# Autodesk Inventor assembly: POM_T5_11
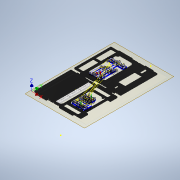
[picture p0: Inventor's stored thumbnail of the model, 180x180]
Saved by Autodesk Inventor 2020 (Build 240168000, 168)
## iProperties
Created: 2021-08-27
Part Number: POM_T5_11
Document SubType Name: Assembly
Designer: Masato
Author: Masato
## Documents named in this file (15)
- C:\Users\L20C1118 森　圭汰\Documents\220428_open\SUSTAINA-OP\Cam\POM_T5_11.iam
- C:\Users\L20C1118 森　圭汰\Documents\220428_open\SUSTAINA-OP\Cam\DisposableBoard.ipt
- C:\Users\L20C1118 森　圭汰\Documents\220428_open\SUSTAINA-OP\UpperBody\Cockpit\Cockpit_carrier_board_frame.ipt
- C:\Users\L20C1118 森　圭汰\Documents\220428_open\SUSTAINA-OP\UpperBody\Cockpit\Cockpit_circuit_board_frame.ipt
- C:\Users\L20C1118 森　圭汰\Documents\220428_open\SUSTAINA-OP\UpperBody\Cockpit\Cockpit_front_frame.ipt
- C:\Users\L20C1118 森　圭汰\Documents\220428_open\SUSTAINA-OP\Jig\Head_horn_frame_Jig.ipt
- C:\Users\L20C1118 森　圭汰\Documents\220428_open\SUSTAINA-OP\UpperBody\Cockpit\Cockpit_back_frame.ipt
- C:\Users\L20C1118 森　圭汰\Documents\220428_open\SUSTAINA-OP\Jig\Cockpit_back_frame_Jig.ipt
- C:\Users\L20C1118 森　圭汰\Documents\220428_open\SUSTAINA-OP\Jig\Cockpit_battery_back_door_Jig.ipt
- C:\Users\L20C1118 森　圭汰\Documents\220428_open\SUSTAINA-OP\Jig\Cockpit_battery_bottom_frame_Jig.ipt
- C:\Users\L20C1118 森　圭汰\Documents\220428_open\SUSTAINA-OP\Jig\Cockpit_battery_bottom_frame_Jig_2.ipt
- C:\Users\L20C1118 森　圭汰\Documents\220428_open\SUSTAINA-OP\Jig\Camera_side_frame_Jig.ipt
- C:\Users\L20C1118 森　圭汰\Documents\220428_open\SUSTAINA-OP\Jig\Head_diagonal_Jig.ipt
- C:\Users\L20C1118 森　圭汰\Documents\220428_open\SUSTAINA-OP\Jig\ForeArm_diagonal_Jig_1.ipt
- C:\Users\L20C1118 森　圭汰\Documents\220428_open\SUSTAINA-OP\Jig\ForeArm_diagonal_Jig_2.ipt
## Components (16 placed, 14 different names)
1. DisposableBoard:1 — メイト:2, メイト:1, フラッシュ:1, フラッシュ:2, メイト:5, メイト:12, フラッシュ:3, フラッシュ:4, メイト:13, メイト:40, メイト:43, メイト:44, メイト:45, メイト:46, メイト:51, メイト:54, メイト:56, メイト:58
2. Cockpit_carrier_board_frame:1 — メイト:5, メイト:15, フラッシュ:6, メイト:38, メイト:41, 正接:2, メイト:49
3. Cockpit_circuit_board_frame:1 — フラッシュ:5, メイト:13, メイト:14, メイト:42, メイト:47, 正接:1, メイト:53
4. Cockpit_front_frame:2 — メイト:12, フラッシュ:3, フラッシュ:4, フラッシュ:5, メイト:14, メイト:15, フラッシュ:6, メイト:39
5. Cockpit_back_frame:1 — メイト:40, メイト:41, メイト:42
6. Cockpit_back_frame_Jig:1 — メイト:43, フラッシュ:7, メイト:48, メイト:52, フラッシュ:10, メイト:57
7. Cockpit_battery_back_door_Jig:1 — メイト:44, メイト:47, 正接:1, フラッシュ:7, メイト:48
8. Cockpit_battery_bottom_frame_Jig:1 — メイト:45, フラッシュ:8, メイト:50, メイト:55, フラッシュ:9
9. Cockpit_battery_bottom_frame_Jig_2:1 — メイト:46, 正接:2, メイト:49, フラッシュ:8, メイト:50
10. Camera_side_frame_Jig:1 — メイト:51, メイト:52, メイト:53
11. Head_diagonal_Jig:1 — メイト:54, メイト:55, フラッシュ:9, フラッシュ:11, メイト:59
12. ForeArm_diagonal_Jig_1:1 — メイト:56, フラッシュ:10, メイト:57
13. ForeArm_diagonal_Jig_2:1 — メイト:58, フラッシュ:11, メイト:59
14. Head_horn_frame_Jig:1 — メイト:37, メイト:38, メイト:39
15. Head_horn_frame_Jig:2
16. Head_horn_frame_Jig:3
## Component patterns: (3 elements, first: Head_horn_frame_Jig:1)
## Relationships (43: Mate 30, Flush 11, Tangent 2)
- メイト:2 [Mate]: DisposableBoard:1
- メイト:1 [Mate]: DisposableBoard:1
- フラッシュ:1 [Flush]: DisposableBoard:1
- フラッシュ:2 [Flush]: DisposableBoard:1
- メイト:5 [Mate]: DisposableBoard:1 ↔ Cockpit_carrier_board_frame:1
- メイト:12 [Mate]: DisposableBoard:1 ↔ Cockpit_front_frame:2
- フラッシュ:3 [Flush] (2.5 mm): DisposableBoard:1 ↔ Cockpit_front_frame:2
- フラッシュ:4 [Flush] (2.5 mm): DisposableBoard:1 ↔ Cockpit_front_frame:2
- フラッシュ:5 [Flush]: Cockpit_circuit_board_frame:1 ↔ Cockpit_front_frame:2
- メイト:13 [Mate]: DisposableBoard:1 ↔ Cockpit_circuit_board_frame:1
- メイト:14 [Mate] (2.5 mm): Cockpit_circuit_board_frame:1 ↔ Cockpit_front_frame:2
- メイト:15 [Mate] (2.5 mm): Cockpit_carrier_board_frame:1 ↔ Cockpit_front_frame:2
- フラッシュ:6 [Flush]: Cockpit_carrier_board_frame:1 ↔ Cockpit_front_frame:2
- メイト:37 [Mate]: Head_horn_frame_Jig:1
- メイト:38 [Mate] (2.5 mm): Cockpit_carrier_board_frame:1 ↔ Head_horn_frame_Jig:1
- メイト:39 [Mate] (5 mm): Cockpit_front_frame:2 ↔ Head_horn_frame_Jig:1
- メイト:40 [Mate]: DisposableBoard:1 ↔ Cockpit_back_frame:1
- メイト:41 [Mate] (2.5 mm): Cockpit_carrier_board_frame:1 ↔ Cockpit_back_frame:1
- メイト:42 [Mate] (2.5 mm): Cockpit_circuit_board_frame:1 ↔ Cockpit_back_frame:1
- メイト:43 [Mate]: DisposableBoard:1 ↔ Cockpit_back_frame_Jig:1
- メイト:44 [Mate]: DisposableBoard:1 ↔ Cockpit_battery_back_door_Jig:1
- メイト:45 [Mate]: DisposableBoard:1 ↔ Cockpit_battery_bottom_frame_Jig:1
- メイト:46 [Mate]: DisposableBoard:1 ↔ Cockpit_battery_bottom_frame_Jig_2:1
- メイト:47 [Mate] (2.5 mm): Cockpit_circuit_board_frame:1 ↔ Cockpit_battery_back_door_Jig:1
- 正接:1 [Tangent] (2.5 mm): Cockpit_circuit_board_frame:1 ↔ Cockpit_battery_back_door_Jig:1
- フラッシュ:7 [Flush]: Cockpit_back_frame_Jig:1 ↔ Cockpit_battery_back_door_Jig:1
- メイト:48 [Mate] (2.5 mm): Cockpit_back_frame_Jig:1 ↔ Cockpit_battery_back_door_Jig:1
- 正接:2 [Tangent] (2.5 mm): Cockpit_carrier_board_frame:1 ↔ Cockpit_battery_bottom_frame_Jig_2:1
- メイト:49 [Mate] (5 mm): Cockpit_carrier_board_frame:1 ↔ Cockpit_battery_bottom_frame_Jig_2:1
- フラッシュ:8 [Flush]: Cockpit_battery_bottom_frame_Jig:1 ↔ Cockpit_battery_bottom_frame_Jig_2:1
- メイト:50 [Mate] (2.5 mm): Cockpit_battery_bottom_frame_Jig:1 ↔ Cockpit_battery_bottom_frame_Jig_2:1
- メイト:51 [Mate]: DisposableBoard:1 ↔ Camera_side_frame_Jig:1
- メイト:52 [Mate] (2.5 mm): Cockpit_back_frame_Jig:1 ↔ Camera_side_frame_Jig:1
- メイト:53 [Mate] (2.5 mm): Cockpit_circuit_board_frame:1 ↔ Camera_side_frame_Jig:1
- メイト:54 [Mate]: DisposableBoard:1 ↔ Head_diagonal_Jig:1
- メイト:55 [Mate] (2.5 mm): Cockpit_battery_bottom_frame_Jig:1 ↔ Head_diagonal_Jig:1
- フラッシュ:9 [Flush]: Cockpit_battery_bottom_frame_Jig:1 ↔ Head_diagonal_Jig:1
- メイト:56 [Mate]: DisposableBoard:1 ↔ ForeArm_diagonal_Jig_1:1
- フラッシュ:10 [Flush]: Cockpit_back_frame_Jig:1 ↔ ForeArm_diagonal_Jig_1:1
- メイト:57 [Mate] (2.5 mm): Cockpit_back_frame_Jig:1 ↔ ForeArm_diagonal_Jig_1:1
- メイト:58 [Mate]: DisposableBoard:1 ↔ ForeArm_diagonal_Jig_2:1
- フラッシュ:11 [Flush]: Head_diagonal_Jig:1 ↔ ForeArm_diagonal_Jig_2:1
- メイト:59 [Mate] (2.5 mm): Head_diagonal_Jig:1 ↔ ForeArm_diagonal_Jig_2:1
